# Autodesk Inventor assembly: цепь_MIR2
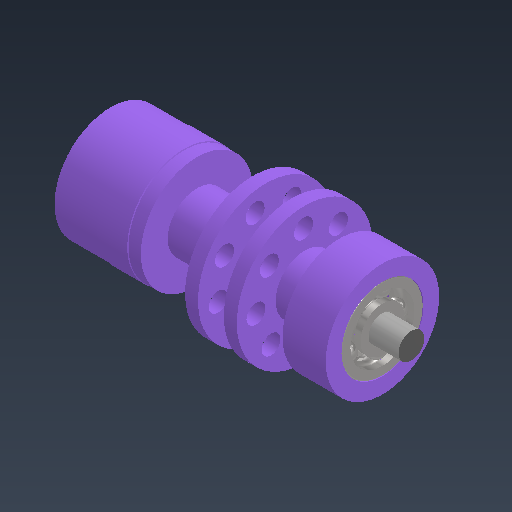
[picture p0: Inventor's stored thumbnail of the model, 512x512]
Saved by Autodesk Inventor 2025 (Build 290162000, 162)
## iProperties
Created: 2024-07-09
Part Number: цепь_MIR2
Document SubType Name: Assembly
Designer: GameHD
Author: Phantom
## Documents named in this file (6)
- C:\Users\GameHD\Desktop\Phantom 16950\цепь_MIR2.iam
- C:\Users\GameHD\Desktop\Phantom 16950\Цепной привод2_MIR2.iam
- C:\Users\GameHD\Desktop\Phantom 16950\втулка для подш 2 часть_MIR4.ipt
- C:\Users\GameHD\Desktop\Phantom 16950\втулка для подш_MIR4.ipt
- C:\Users\GameHD\Desktop\Phantom 16950\Деталь_64_MIR4.ipt
- C:\Users\GameHD\Desktop\Phantom 16950\BS 290 SKF - SKF 626-RZ_MIR4.ipt
## Components (6 placed, 5 different names)
1. Цепной привод2_MIR2:1 [sub-assembly] — Заподлицо:4, Совмещение:24, Совмещение:22
2. втулка для подш 2 часть_MIR4:1 — Совмещение:16, Совмещение:23, Совмещение:20
3. втулка для подш_MIR4:1 — Заподлицо:4, Совмещение:24, Совмещение:22, Совмещение:16, Совмещение:17, Совмещение:18
4. Деталь_64_MIR4:1 — Совмещение:23, Совмещение:17, Совмещение:21, Совмещение:19
5. BS 290 SKF - SKF 626-RZ_MIR4:1 — Совмещение:21, Совмещение:20
6. BS 290 SKF - SKF 626-RZ_MIR4:2 — Совмещение:19, Совмещение:18
## Relationships (10: Mate 9, Flush 1)
- Заподлицо:4 [Flush] (4 mm): Цепной привод2_MIR2:1 ↔ втулка для подш_MIR4:1
- Совмещение:24 [Mate]: Цепной привод2_MIR2:1 ↔ втулка для подш_MIR4:1
- Совмещение:22 [Mate]: Цепной привод2_MIR2:1 ↔ втулка для подш_MIR4:1
- Совмещение:16 [Mate]: втулка для подш 2 часть_MIR4:1 ↔ втулка для подш_MIR4:1
- Совмещение:23 [Mate]: втулка для подш 2 часть_MIR4:1 ↔ Деталь_64_MIR4:1
- Совмещение:17 [Mate]: втулка для подш_MIR4:1 ↔ Деталь_64_MIR4:1
- Совмещение:21 [Mate]: Деталь_64_MIR4:1 ↔ BS 290 SKF - SKF 626-RZ_MIR4:1
- Совмещение:20 [Mate]: втулка для подш 2 часть_MIR4:1 ↔ BS 290 SKF - SKF 626-RZ_MIR4:1
- Совмещение:19 [Mate]: Деталь_64_MIR4:1 ↔ BS 290 SKF - SKF 626-RZ_MIR4:2
- Совмещение:18 [Mate]: втулка для подш_MIR4:1 ↔ BS 290 SKF - SKF 626-RZ_MIR4:2
